# Autodesk Inventor assembly: Final Assembly
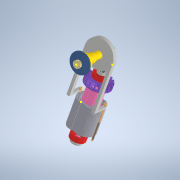
[picture p0: Inventor's stored thumbnail of the model, 180x180]
Saved by Autodesk Inventor 2022 (Build 260153000, 153)
## iProperties
Created: 2023-04-24
Part Number: Final Assembly
Document SubType Name: Assembly
Designer: aibad
Author: aibad
## Documents named in this file (16)
- C:\Users\aibad\Desktop\Enginnering Graphics (ME-2207)\Final Project\Final Assembly.iam
- C:\Users\aibad\Desktop\Enginnering Graphics (ME-2207)\Final Project\Aemature Final.ipt
- C:\Users\aibad\Desktop\Enginnering Graphics (ME-2207)\Final Project\Bearing 6000.ipt
- C:\Users\aibad\Desktop\Enginnering Graphics (ME-2207)\Final Project\Bushing.ipt
- C:\Users\aibad\Desktop\Enginnering Graphics (ME-2207)\Final Project\Chassis.ipt
- C:\Users\aibad\Desktop\Enginnering Graphics (ME-2207)\Final Project\Clip.ipt
- C:\Users\aibad\Desktop\Enginnering Graphics (ME-2207)\Final Project\Fan (Completed).ipt
- C:\Users\aibad\Desktop\Enginnering Graphics (ME-2207)\Final Project\Fan Shaft.ipt
- C:\Users\aibad\Desktop\Enginnering Graphics (ME-2207)\Final Project\Fork.ipt
- C:\Users\aibad\Desktop\Enginnering Graphics (ME-2207)\Final Project\Spindle.ipt
- C:\Users\aibad\Desktop\Enginnering Graphics (ME-2207)\Final Project\Stator Final Project.ipt
- C:\Users\aibad\Desktop\Enginnering Graphics (ME-2207)\Final Project\Washer (Finished).ipt
- C:\Users\aibad\Desktop\Enginnering Graphics (ME-2207)\Final Project\Bearing 626.ipt
- C:\Users\aibad\Desktop\Enginnering Graphics (ME-2207)\Final Project\Cap Screw.ipt
- C:\Users\aibad\Desktop\Enginnering Graphics (ME-2207)\Final Project\Assembly1.iam
- C:\Users\aibad\Desktop\Enginnering Graphics (ME-2207)\Final Project\Long Screw.ipt
## Components (19 placed, 15 different names)
1. Aemature Final:1 — Rotational:1, Insert:1, Rigid:3, Rigid:4
2. Bearing 6000:2 — Rigid:1, Insert:3
3. Bushing:2 — Rotational:7
4. Chassis:2 — Insert:2, Rotational:6, Rigid:2, Rotational:10
5. Clip:1 — Rotational:4
6. Fan (Completed):1 — Rotational:2
7. Fan Shaft:1 — Insert:1, Rotational:2, Rigid:1, Rotational:3, Rotational:4
8. Spindle:1 — Insert:2, Rotational:5, Rotational:7, Rotational:8, Rotational:9
9. Washer (Finished):1 — Rotational:5
10. Stator Final Project:4 — Rotational:1, Rigid:2, Insert:6
11. Bearing 626:1 — Insert:3
12. Cap Screw:1 — Rotational:9
13. Assembly1:1 [sub-assembly] — Rotational:3, Tangent:1
14. Bearing 6000:3 — Rotational:6
15. Long Screw:1 — Insert:6
16. Long Screw:2 — Rotational:10
17. Bearing 6000:4 — Rigid:3
18. Bearing 626:2 — Rigid:4
19. Fork:1 — Rotational:8, Tangent:1
## Relationships (19: RevoluteJoint 10, Insert 4, WeldJoint 4, Tangent 1)
- Rotational:1 [RevoluteJoint] (-60 mm): Aemature Final:1 ↔ Stator Final Project:4
- Insert:1: Aemature Final:1 ↔ Fan Shaft:1
- Rotational:2 [RevoluteJoint]: Fan (Completed):1 ↔ Fan Shaft:1
- Insert:2 (-30 mm): Chassis:2 ↔ Spindle:1
- Rigid:1 [WeldJoint] (2 mm): Bearing 6000:2 ↔ Fan Shaft:1
- Insert:3 (-1 mm): Bearing 6000:2 ↔ Bearing 626:1
- Rotational:3 [RevoluteJoint] (5 mm): Fan Shaft:1 ↔ Assembly1:1
- Rotational:4 [RevoluteJoint]: Clip:1 ↔ Fan Shaft:1
- Rotational:5 [RevoluteJoint]: Spindle:1 ↔ Washer (Finished):1
- Rotational:6 [RevoluteJoint] (-2.5 mm): Chassis:2 ↔ Bearing 6000:3
- Rotational:7 [RevoluteJoint] (-9 mm): Bushing:2 ↔ Spindle:1
- Rigid:2 [WeldJoint] (5 mm): Chassis:2 ↔ Stator Final Project:4
- Rigid:3 [WeldJoint] (12 mm): Aemature Final:1 ↔ Bearing 6000:4
- Rigid:4 [WeldJoint] (12 mm): Aemature Final:1 ↔ Bearing 626:2
- Insert:6 (7 mm): Stator Final Project:4 ↔ Long Screw:1
- Rotational:8 [RevoluteJoint] (10 mm): Spindle:1 ↔ Fork:1
- Tangent:1: Assembly1:1 ↔ Fork:1
- Rotational:9 [RevoluteJoint] (-8 mm): Spindle:1 ↔ Cap Screw:1
- Rotational:10 [RevoluteJoint] (59 mm): Chassis:2 ↔ Long Screw:2
